# Autodesk Inventor assembly: Leg Asswmbly
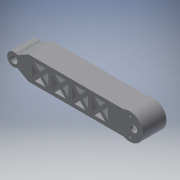
[picture p0: Inventor's stored thumbnail of the model, 180x180]
Saved by Autodesk Inventor 2018.2 (Build 222227000, 227)
## iProperties
Created: 2018-02-09
Part Number: Leg Asswmbly
Document SubType Name: Assembly
Designer: MIABo
Mass: 210.05 g
Surface Area: 665.262 cm^2
Volume: 210.05 cm^3
Density: 1 g/cm^3
Author: MIABo
## Documents named in this file (3)
- C:\Users\MIABo\OneDrive\Documents\GitHub\Ares\Leg Asswmbly.iam
- C:\Users\MIABo\OneDrive\Documents\GitHub\Ares\Leg Box.ipt
- C:\Users\MIABo\OneDrive\Documents\GitHub\Ares\Suspension Bracket Mount.ipt
## Components (2 placed, 2 different names)
1. Leg Box:1 — Mate:1, Mate:2
2. Suspension Bracket Mount:1 — Mate:1, Mate:2
## Relationships (2: Mate 2)
- Mate:1: Leg Box:1 ↔ Suspension Bracket Mount:1
- Mate:2: Leg Box:1 ↔ Suspension Bracket Mount:1
